# Autodesk Inventor assembly: BatteryRack-Assembly-Stack
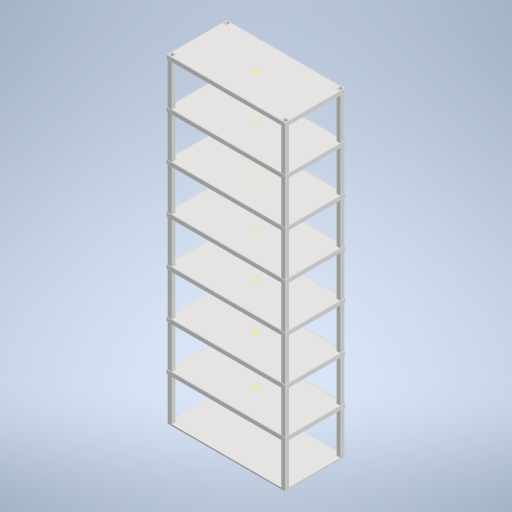
[picture p0: Inventor's stored thumbnail of the model, 512x512]
Saved by Autodesk Inventor 2023 (Build 270158000, 158)
## iProperties
Created: 2023-06-24
Part Number: BatteryRack-Assembly-Stack
Document SubType Name: Assembly
Designer: incep
Author: incep
## Documents named in this file (6)
- C:\Projects\TechnoGecko\TechnoGecko-BatteryRack\BatteryRack-Assembly-Stack.iam
- C:\Projects\TechnoGecko\TechnoGecko-BatteryRack\assyBase.ipt
- C:\Projects\TechnoGecko\TechnoGecko-BatteryRack\vertical.ipt
- C:\Projects\TechnoGecko\TechnoGecko-BatteryRack\beamX.ipt
- C:\Projects\TechnoGecko\TechnoGecko-BatteryRack\beamZ.ipt
- C:\Projects\TechnoGecko\TechnoGecko-BatteryRack\shelf.ipt
## Components (64 placed, 5 different names)
1. assyBase:1 — Mate:1, Mate:2, Mate:3, Mate:4, Flush:1, Flush:2, Mate:5, Mate:6, Flush:3, Flush:4, Mate:7, Flush:5, Flush:6, Mate:8, Flush:7, Flush:8
2. vertical:1 — Flush:1, Flush:2, Mate:5, Flush:10, Mate:12, Flush:11
3. vertical:2 — Mate:6, Flush:3, Flush:4, Flush:9, Mate:9, Mate:10, Mate:11, Mate:15, Mate:16, Mate:17
4. vertical:3 — Mate:7, Flush:5, Flush:6, Mate:19, Mate:20
5. vertical:4 — Mate:8, Flush:7, Flush:8, Mate:13, Mate:14, Flush:12, Mate:18
6. beamX:1 — Flush:9, Mate:9, Mate:10, Mate:11
7. beamX:2 — Flush:10, Mate:12, Mate:13, Mate:14, Mate:23
8. beamZ:1 — Flush:11, Mate:15, Mate:16, Mate:17, Mate:21
9. beamZ:2 — Flush:12, Mate:18, Mate:19, Mate:20, Mate:22
10. shelf:1 — Mate:21, Mate:22, Mate:23
11. vertical:5
12. vertical:6
13. vertical:7
14. vertical:8
15. beamX:3
16. beamX:4
17. beamZ:3
18. beamZ:4
19. shelf:2
20. vertical:9
21. vertical:10
22. vertical:11
23. vertical:12
24. beamX:5
25. beamX:6
26. beamZ:5
27. beamZ:6
28. shelf:3
29. vertical:13
30. vertical:14
31. vertical:15
32. vertical:16
33. beamX:7
34. beamX:8
35. beamZ:7
36. beamZ:8
37. shelf:4
38. vertical:17
39. vertical:18
40. vertical:19
41. vertical:20
42. beamX:9
43. beamX:10
44. beamZ:9
45. beamZ:10
46. shelf:5
47. vertical:21
48. vertical:22
49. vertical:23
50. vertical:24
51. beamX:11
52. beamX:12
53. beamZ:11
54. beamZ:12
55. shelf:6
56. vertical:25
57. vertical:26
58. vertical:27
59. vertical:28
60. beamX:13
61. beamX:14
62. beamZ:13
63. beamZ:14
64. shelf:7
## Component patterns: (7 elements, first: vertical:1 + vertical:2 + vertical:3 + vertical:4 + beamX:1 + beamX:2 + beamZ:1 + beamZ:2 + shelf:1)
## Relationships (35: Mate 23, Flush 12)
- Mate:1: assyBase:1
- Mate:2: assyBase:1
- Mate:3: assyBase:1
- Mate:4: assyBase:1
- Flush:1: assyBase:1 ↔ vertical:1
- Flush:2: assyBase:1 ↔ vertical:1
- Mate:5: assyBase:1 ↔ vertical:1
- Mate:6: assyBase:1 ↔ vertical:2
- Flush:3: assyBase:1 ↔ vertical:2
- Flush:4: assyBase:1 ↔ vertical:2
- Mate:7: assyBase:1 ↔ vertical:3
- Flush:5: assyBase:1 ↔ vertical:3
- Flush:6: assyBase:1 ↔ vertical:3
- Mate:8: assyBase:1 ↔ vertical:4
- Flush:7: assyBase:1 ↔ vertical:4
- Flush:8: assyBase:1 ↔ vertical:4
- Flush:9: vertical:2 ↔ beamX:1
- Mate:9: vertical:2 ↔ beamX:1
- Mate:10: vertical:2 ↔ beamX:1
- Mate:11: vertical:2 ↔ beamX:1
- Flush:10: vertical:1 ↔ beamX:2
- Mate:12: vertical:1 ↔ beamX:2
- Mate:13: vertical:4 ↔ beamX:2
- Mate:14: vertical:4 ↔ beamX:2
- Flush:11: vertical:1 ↔ beamZ:1
- Mate:15: vertical:2 ↔ beamZ:1
- Mate:16: vertical:2 ↔ beamZ:1
- Mate:17: vertical:2 ↔ beamZ:1
- Flush:12: vertical:4 ↔ beamZ:2
- Mate:18: vertical:4 ↔ beamZ:2
- Mate:19: vertical:3 ↔ beamZ:2
- Mate:20: vertical:3 ↔ beamZ:2
- Mate:21: beamZ:1 ↔ shelf:1
- Mate:22 (1 mm): beamZ:2 ↔ shelf:1
- Mate:23 (1 mm): beamX:2 ↔ shelf:1
